# Autodesk Inventor assembly: 100-10-FRAME-DIFFERENTIAL-REINF-02
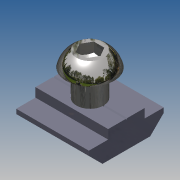
[picture p0: Inventor's stored thumbnail of the model, 180x180]
Saved by Autodesk Inventor 2018.2 (Build 222227000, 227)
## iProperties
Manager: feesmrt
Company: FRANCOR
Part Number: 100-10-FRAME-DIFFERENTIAL-REINF-02
Project: Rescue Robot
Cost Center: -
Material: Generisch
Document SubType Name: Assembly
Designer: feesmrt
Engineer: feesmrt
Authority: feesmrt
Description: Verbinder Differential Verstärkungsblech
Stock Number: 100-10-FRAME-DIFFERENTIAL-REINF-02
Subject: Rescue Robot
Author: feesmrt
Revision Number: 1
Title: Verbinder Differential Verstärkungsblech
## Documents named in this file (3)
- C:\Users\feesmrt\Documents\FRANC0R\CAD\02-Rocker-Bogie-Robot\100-CHASSIS\10-FRAME\100-10-FRAME-DIFFERENTIAL-REINF-02.iam
- C:\Users\feesmrt\Documents\FRANC0R\CAD\02-Rocker-Bogie-Robot\900-COMPONENTS\900-50-PROFILES\900-50-PROFILES-CONN-N8xM6.ipt
- C:\Users\feesmrt\Documents\FRANC0R\CAD\02-Rocker-Bogie-Robot\900-COMPONENTS\900-40-SCREWS\900-40-SCREWS-ISO7830_M6x12.ipt
## Components (2 placed, 2 different names)
1. 900-50-PROFILES-CONN-N8xM6:1 — Passend:1, Passend:2
2. 900-40-SCREWS-ISO7830_M6x12:1 — Passend:1, Passend:2
## Relationships (2: Mate 2)
- Passend:1 [Mate] (7.8 mm): 900-50-PROFILES-CONN-N8xM6:1 ↔ 900-40-SCREWS-ISO7830_M6x12:1
- Passend:2 [Mate]: 900-50-PROFILES-CONN-N8xM6:1 ↔ 900-40-SCREWS-ISO7830_M6x12:1
